# Autodesk Inventor assembly: Manillar_freno
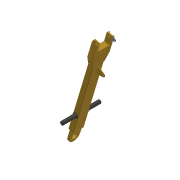
[picture p0: Inventor's stored thumbnail of the model, 180x180]
Saved by Autodesk Inventor 2020 (Build 240168000, 168)
## iProperties
Created: 2020-02-07
Part Number: Manillar_freno
Document SubType Name: Assembly
Designer: Juan Carlos Botero
Mass: 10801.8 g
Surface Area: 7225.8 cm^2
Volume: 1379.7 cm^3
Density: 7.82913 g/cm^3
Author: Juan Carlos Botero
## Documents named in this file (3)
- D:\Drives\OneDrive\Carlos_2\02 TRABAJOS\MULTIPLO\Conveyor\ENSAMBLE\Manillar_freno.iam
- D:\Drives\OneDrive\Carlos_2\02 TRABAJOS\MULTIPLO\Conveyor\ENSAMBLE\Solid2.ipt
- D:\Drives\OneDrive\Carlos_2\02 TRABAJOS\MULTIPLO\Conveyor\ENSAMBLE\manillar tiro.iam
## Components (2 placed, 2 different names)
1. Solid2:1 — Mate:1, Flush:1, Mate:2
2. manillar tiro:1 [sub-assembly] — Mate:1, Flush:1, Mate:2
## Relationships (3: Mate 2, Flush 1)
- Mate:1: Solid2:1 ↔ manillar tiro:1
- Flush:1 (10 mm): Solid2:1 ↔ manillar tiro:1
- Mate:2: Solid2:1 ↔ manillar tiro:1
